# Autodesk Inventor assembly: Right Hook Whole Assembly_v2
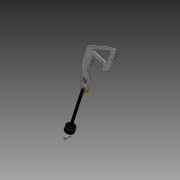
[picture p0: Inventor's stored thumbnail of the model, 180x180]
Saved by Autodesk Inventor 2014 SP1 (Build 180222100, 222)
## iProperties
Created: 2013-03-16
Part Number: Right Hook Whole Assembly_v2
Document SubType Name: Assembly
Designer: Arpan
Mass: 1403.84 g
Surface Area: 1553.7 cm^2
Volume: 264.387 cm^3
Density: 5.30978 g/cm^3
Author: Arpan
## Documents named in this file (4)
- C:\Users\Moses\Documents\Inventor\Sally Rebuild\Rebuild Sally\Right Hook Whole Assembly_v2.iam
- C:\Users\Moses\Documents\Inventor\Sally Rebuild\Rebuild Sally\Right Hook Encoder Assembly.iam
- C:\Users\Moses\Documents\Inventor\Sally Rebuild\Rebuild Sally\Ninja cylinder support bracket.ipt
- C:\Users\Moses\Documents\Inventor\Sally Rebuild\Rebuild Sally\Piston Bracket Assembly - R.iam
## Components (3 placed, 3 different names)
1. Right Hook Encoder Assembly:1 [sub-assembly] — Mate:8, Mate:9, Mate:10
2. Piston Bracket Assembly - R:1 [sub-assembly] — Mate:4, Mate:5, Mate:6, Flush:1, Mate:8, Mate:9, Mate:10
3. Ninja cylinder support bracket:1 — Mate:4, Mate:5, Mate:6, Flush:1
## Relationships (7: Mate 6, Flush 1)
- Mate:4: Piston Bracket Assembly - R:1 ↔ Ninja cylinder support bracket:1
- Mate:5: Piston Bracket Assembly - R:1 ↔ Ninja cylinder support bracket:1
- Mate:6: Piston Bracket Assembly - R:1 ↔ Ninja cylinder support bracket:1
- Flush:1: Piston Bracket Assembly - R:1 ↔ Ninja cylinder support bracket:1
- Mate:8: Right Hook Encoder Assembly:1 ↔ Piston Bracket Assembly - R:1
- Mate:9: Right Hook Encoder Assembly:1 ↔ Piston Bracket Assembly - R:1
- Mate:10: Right Hook Encoder Assembly:1 ↔ Piston Bracket Assembly - R:1
